# Autodesk Inventor assembly: Full Basic Assembly--v2
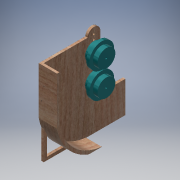
[picture p0: Inventor's stored thumbnail of the model, 180x180]
Saved by Autodesk Inventor 2019 (Build 230136000, 136)
## iProperties
Created: 2019-01-23
Part Number: Full Basic Assembly--v2
Document SubType Name: Assembly
Designer: scigu
Author: scigu
## Documents named in this file (3)
- C:\Users\scigu\Documents\School 18-19\SeCon\Intake\Full Basic Assembly--v2.iam
- C:\Users\scigu\Documents\School 18-19\SeCon\Intake\Wall--v1.ipt
- C:\Users\scigu\Documents\School 18-19\SeCon\Intake\Sprocket.ipt
## Components (3 placed, 2 different names)
1. Wall--v1:1 — Insert:1, Insert:2
2. Sprocket:1 — Insert:1
3. Sprocket:2 — Insert:2
## Relationships (2: Insert 2)
- Insert:1: Wall--v1:1 ↔ Sprocket:1
- Insert:2: Wall--v1:1 ↔ Sprocket:2
